# Autodesk Inventor assembly: coffeeMaker
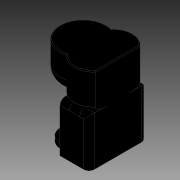
[picture p0: Inventor's stored thumbnail of the model, 180x180]
Saved by Autodesk Inventor 2014 (Build 180170000, 170)
## iProperties
Created: 2014-07-25
Part Number: coffeeMaker
Document SubType Name: Assembly
Designer: hatakeyama
Author: hatakeyama
## Documents named in this file (2)
- C:\Users\hatakeyama\Desktop\homeroom\coffeeMaker.iam
- C:\Users\hatakeyama\Desktop\homeroom\インポートされたコンポーネント\coffeeMaker\coffeeMaker.ipt
## Components (1 placed, 1 different names)
1. coffeeMaker:1 — メイト:1, 角度:1, メイト:2
## Relationships (3: Mate 2, Angle 1)
- メイト:1 [Mate]: coffeeMaker:1
- 角度:1 [Angle] (0 deg): coffeeMaker:1
- メイト:2 [Mate]: coffeeMaker:1
